# Autodesk Inventor assembly: leg_1
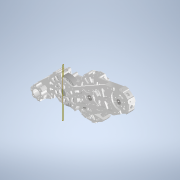
[picture p0: Inventor's stored thumbnail of the model, 180x180]
Saved by Autodesk Inventor 2020 (Build 240168000, 168)
## iProperties
Created: 2020-07-04
Part Number: leg_1
Document SubType Name: Assembly
Designer: psrobotics
Author: psrobotics
## Documents named in this file (25)
- D:\projects-3\biped_gen1\sim\model\leg_2dof_urdf\leg_1.iam
- D:\projects-3\biped_gen1\hardware\90_motor.iam
- D:\projects-3\biped_gen1\hardware\xl_20.ipt
- D:\projects-3\biped_gen1\hardware\xl_wheel_ass.iam
- D:\projects-3\biped_gen1\hardware\shell_2.ipt
- D:\projects-3\biped_gen1\hardware\shell_3.ipt
- D:\projects-3\biped_gen1\hardware\shell_4.ipt
- D:\projects-3\biped_gen1\hardware\motor_h_1.ipt
- D:\projects-3\biped_gen1\hardware\shell_5.ipt
- D:\projects-3\biped_gen1\hardware\bearing_shell_1.ipt
- D:\projects-3\biped_gen1\hardware\bearing_shell_2.ipt
- D:\projects-3\biped_gen1\hardware\xl_30_1.ipt
- D:\projects-3\biped_gen1\hardware\motor_h_4.ipt
- D:\projects-3\biped_gen1\hardware\motor_h_3_m.ipt
- D:\projects-3\biped_gen1\hardware\motor_h_5_m.ipt
- D:\projects-3\biped_gen1\hardware\bearing_35_44_5.ipt
- D:\projects-3\biped_gen1\hardware\end_holder_1.ipt
- D:\projects-3\biped_gen1\hardware\motor_r_1.ipt
- D:\projects-3\biped_gen1\hardware\bearing_8_16_5.ipt
- D:\projects-3\biped_gen1\hardware\bearing_6_13_5.ipt
- D:\projects-3\biped_gen1\hardware\leg_fixer_1.ipt
- D:\projects-3\biped_gen1\hardware\bearing_shell_3.ipt
- D:\projects-3\biped_gen1\hardware\joint_connector_1.ipt
- D:\projects-3\biped_gen1\hardware\joint_connector_2.ipt
- D:\projects-3\biped_gen1\hardware\leg_fixer_2.ipt
## Components (31 placed, 24 different names)
1. 90_motor:1 [sub-assembly] — Insert:1, Insert:2, Flush:4, Insert:58, Insert:59
2. xl_20:1 — Insert:1, Insert:2, Flush:1, Tangent:1
3. xl_wheel_ass:1 [sub-assembly] — Flush:1, Tangent:1, Insert:9
4. shell_2:1 — Angle:1, Insert:9, Insert:18
5. shell_2:3 — Angle:1, Angle:2, Insert:14, Insert:17
6. shell_2:4 — Angle:2, Flush:6, Insert:15, Insert:16, Insert:33, Insert:34
7. shell_3:1 — Flush:4, Flush:5, Insert:25, Insert:26, Insert:42, Insert:43
8. shell_4:1 — Flush:5, Insert:25, Insert:26, Flush:12, Insert:40, Insert:41
9. motor_h_1:1 — Flush:6, Insert:14, Insert:15, Insert:16, Insert:17, Insert:18, Flush:10, Insert:27, Insert:28, Insert:30, Insert:31, Insert:52, Insert:53
10. shell_5:1 — Insert:35, Insert:36, Insert:37, Insert:38
11. bearing_shell_2:1 — Flush:10, Insert:27, Insert:28, Insert:51
12. xl_wheel_ass:2 [sub-assembly] — Insert:32
13. xl_30_1:1 — Insert:46, Flush:13, Flush:14
14. bearing_shell_1:1 — Insert:30, Insert:31, Insert:32
15. motor_h_4:1 — Insert:33, Insert:34, Insert:37, Insert:38, Insert:45, Insert:49, Insert:50, Insert:54, Flush:16, Insert:56, Insert:57, Insert:73, Insert:74
16. motor_h_3_m:1 — Insert:35, Insert:36, Insert:42, Insert:43, Flush:15, Insert:47, Insert:48, Insert:58, Insert:59, Flush:18, Insert:63, Insert:64, Flush:19, Insert:65, Insert:66
17. motor_h_5_m:1 — Flush:12, Insert:40, Insert:41
18. bearing_35_44_5:1 — Insert:45, Insert:46
19. end_holder_1:1 — Flush:13, Flush:14, Insert:49, Insert:50, Insert:55
20. motor_r_1:1 — Flush:15, Insert:47, Insert:48, Flush:17, Insert:60, Insert:61
21. bearing_8_16_5:1 — Insert:55
22. bearing_8_16_5:2 — Insert:52
23. bearing_8_16_5:3 — Insert:54
24. bearing_8_16_5:4 — Insert:53
25. bearing_6_13_5:1 — Insert:51
26. leg_fixer_1:1 — Flush:16, Insert:56, Insert:57
27. bearing_shell_3:1 — Flush:17, Insert:60, Insert:61, Insert:62
28. bearing_8_16_5:5 — Insert:62
29. joint_connector_1:1 — Flush:18, Insert:63, Insert:64
30. joint_connector_2:1 — Flush:19, Insert:65, Insert:66
31. leg_fixer_2:1 — Insert:73, Insert:74
## Relationships (65: Insert 49, Flush 13, Angle 2, Tangent 1)
- Insert:1: 90_motor:1 ↔ xl_20:1
- Insert:2: 90_motor:1 ↔ xl_20:1
- Flush:1: xl_20:1 ↔ xl_wheel_ass:1
- Tangent:1 (1.3 mm): xl_20:1 ↔ xl_wheel_ass:1
- Angle:1 (160 deg): shell_2:1 ↔ shell_2:3
- Angle:2 (230 deg): shell_2:3 ↔ shell_2:4
- Insert:9 (-0.5 mm): xl_wheel_ass:1 ↔ shell_2:1
- Flush:4: 90_motor:1 ↔ shell_3:1
- Flush:5: shell_3:1 ↔ shell_4:1
- Flush:6: shell_2:4 ↔ motor_h_1:1
- Insert:14: shell_2:3 ↔ motor_h_1:1
- Insert:15: shell_2:4 ↔ motor_h_1:1
- Insert:16: shell_2:4 ↔ motor_h_1:1
- Insert:17: shell_2:3 ↔ motor_h_1:1
- Insert:18: shell_2:1 ↔ motor_h_1:1
- Insert:25: shell_3:1 ↔ shell_4:1
- Insert:26: shell_3:1 ↔ shell_4:1
- Flush:10: motor_h_1:1 ↔ bearing_shell_2:1
- Insert:27: motor_h_1:1 ↔ bearing_shell_2:1
- Insert:28: motor_h_1:1 ↔ bearing_shell_2:1
- Insert:30: motor_h_1:1 ↔ bearing_shell_1:1
- Insert:31: motor_h_1:1 ↔ bearing_shell_1:1
- Insert:32: xl_wheel_ass:2 ↔ bearing_shell_1:1
- Insert:33: shell_2:4 ↔ motor_h_4:1
- Insert:34: shell_2:4 ↔ motor_h_4:1
- Insert:35: shell_5:1 ↔ motor_h_3_m:1
- Insert:36: shell_5:1 ↔ motor_h_3_m:1
- Insert:37: shell_5:1 ↔ motor_h_4:1
- Insert:38: shell_5:1 ↔ motor_h_4:1
- Flush:12: shell_4:1 ↔ motor_h_5_m:1
- Insert:40: shell_4:1 ↔ motor_h_5_m:1
- Insert:41: shell_4:1 ↔ motor_h_5_m:1
- Insert:42: shell_3:1 ↔ motor_h_3_m:1
- Insert:43: shell_3:1 ↔ motor_h_3_m:1
- Insert:45: motor_h_4:1 ↔ bearing_35_44_5:1
- Insert:46: xl_30_1:1 ↔ bearing_35_44_5:1
- Flush:13: xl_30_1:1 ↔ end_holder_1:1
- Flush:14 (1 mm): xl_30_1:1 ↔ end_holder_1:1
- Flush:15: motor_h_3_m:1 ↔ motor_r_1:1
- Insert:47: motor_h_3_m:1 ↔ motor_r_1:1
- Insert:48: motor_h_3_m:1 ↔ motor_r_1:1
- Insert:49: motor_h_4:1 ↔ end_holder_1:1
- Insert:50: motor_h_4:1 ↔ end_holder_1:1
- Insert:51: bearing_shell_2:1 ↔ bearing_6_13_5:1
- Insert:52: motor_h_1:1 ↔ bearing_8_16_5:2
- Insert:53: motor_h_1:1 ↔ bearing_8_16_5:4
- Insert:54: motor_h_4:1 ↔ bearing_8_16_5:3
- Insert:55: end_holder_1:1 ↔ bearing_8_16_5:1
- Flush:16: motor_h_4:1 ↔ leg_fixer_1:1
- Insert:56: motor_h_4:1 ↔ leg_fixer_1:1
- Insert:57: motor_h_4:1 ↔ leg_fixer_1:1
- Insert:58: 90_motor:1 ↔ motor_h_3_m:1
- Insert:59: 90_motor:1 ↔ motor_h_3_m:1
- Flush:17: motor_r_1:1 ↔ bearing_shell_3:1
- Insert:60: motor_r_1:1 ↔ bearing_shell_3:1
- Insert:61: motor_r_1:1 ↔ bearing_shell_3:1
- Insert:62: bearing_shell_3:1 ↔ bearing_8_16_5:5
- Flush:18: motor_h_3_m:1 ↔ joint_connector_1:1
- Insert:63: motor_h_3_m:1 ↔ joint_connector_1:1
- Insert:64: motor_h_3_m:1 ↔ joint_connector_1:1
- Flush:19: motor_h_3_m:1 ↔ joint_connector_2:1
- Insert:65: motor_h_3_m:1 ↔ joint_connector_2:1
- Insert:66: motor_h_3_m:1 ↔ joint_connector_2:1
- Insert:73: motor_h_4:1 ↔ leg_fixer_2:1
- Insert:74: motor_h_4:1 ↔ leg_fixer_2:1
